# Autodesk Inventor assembly: ALFA1
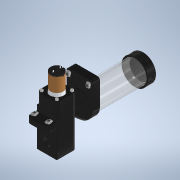
[picture p0: Inventor's stored thumbnail of the model, 180x180]
Saved by Autodesk Inventor 2020.2 (Build 242310000, 310)
## iProperties
Created: 2020-11-09
Part Number: ALFA1
Document SubType Name: Assembly
Designer: JK
Author: JK
## Documents named in this file (15)
- C:\Users\JK\Documents\Inventor\BioMixer\DispensadorPolvo\DispensadordePolvo.iam
- C:\Users\JK\Documents\Inventor\BioMixer\DispensadorPolvo\JGA25-372 24V Motor.ipt
- C:\Users\JK\Documents\Inventor\BioMixer\DispensadorPolvo\Bearing.ipt
- C:\Users\JK\Documents\Inventor\BioMixer\DispensadorPolvo\soportemotor.ipt
- C:\Users\JK\Documents\Inventor\BioMixer\DispensadorPolvo\taparodamiento.ipt
- C:\Users\JK\Documents\Inventor\BioMixer\DispensadorPolvo\TornilloDCGrande.ipt
- C:\Users\JK\Documents\Inventor\BioMixer\DispensadorPolvo\Conjuntocontenedor.iam
- C:\Users\JK\Documents\Inventor\BioMixer\DispensadorPolvo\PernoM5x15Plano.ipt
- C:\Users\JK\Documents\Inventor\BioMixer\DispensadorPolvo\TuercaTM5Perfil2020.ipt
- C:\Users\JK\Documents\Inventor\BioMixer\DispensadorPolvo\BarrilDispensador.ipt
- C:\Users\JK\Documents\Inventor\BioMixer\DispensadorPolvo\PernoM3x6Avellanado.ipt
- C:\Users\JK\Documents\Inventor\BioMixer\DispensadorPolvo\TuercaM3.ipt
- C:\Users\JK\Documents\Inventor\BioMixer\DispensadorPolvo\PernoM3x10Parker.ipt
- C:\Users\JK\Documents\Inventor\BioMixer\DispensadorPolvo\PernoM3x30Parker.ipt
- C:\Users\JK\Documents\Inventor\BioMixer\DispensadorPolvo\PrisioneroM3x6.ipt
## Components (31 placed, 14 different names)
1. JGA25-372 24V Motor:1 — Mate:17, Mate:18, Mate:19, Mate:22, Mate:27, Mate:30, Mate:31, Mate:39, Mate:40, Mate:59
2. BarrilDispensador:1 — Mate:25, Mate:26, Mate:27, Mate:28, Mate:29, Flush:1, Mate:32, Mate:33, Mate:34, Mate:35, Angle:2, Angle:3, Mate:38, Flush:5, Angle:4, Angle:5, Angle:6, Angle:7, Angle:8, Angle:9, Angle:10, Angle:11, Mate:49, Mate:50
3. Bearing:1 — Mate:25, Mate:26
4. soportemotor:1 — Mate:17, Mate:18, Mate:19, Mate:29, Flush:1, Angle:1, Flush:6, Flush:7, Mate:60, Mate:61
5. taparodamiento:1 — Mate:22, Mate:28, Flush:5, Mate:41, Mate:42, Mate:43, Mate:44, Mate:46, Mate:47, Mate:48, Mate:51, Mate:52, Mate:53, Mate:54, Mate:55
6. TornilloDCGrande:1 — Mate:30, Mate:31, Mate:56, Angle:12, Mate:58
7. Conjuntocontenedor:1 [sub-assembly] — Mate:32, Angle:1
8. PernoM5x15Plano:1 — Mate:34, Flush:3, Mate:37
9. PernoM5x15Plano:2 — Mate:33, Flush:3, Mate:35, Mate:36
10. TuercaTM5Perfil2020:1 — Mate:36, Angle:2, Flush:4, Mate:38
11. TuercaTM5Perfil2020:2 — Mate:37, Angle:3, Flush:4
12. PernoM3x6Avellanado:1 — Mate:39, Flush:6
13. PernoM3x6Avellanado:2 — Mate:40, Flush:7
14. TuercaM3:1 — Mate:43, Angle:6, Flush:10
15. TuercaM3:2 — Angle:9, Flush:11, Mate:47, Mate:49
16. TuercaM3:3 — Mate:44, Angle:7, Flush:9, Mate:50
17. TuercaM3:4 — Angle:10, Flush:13, Mate:48
18. TuercaM3:5 — Angle:11, Flush:12, Mate:46
19. TuercaM3:6 — Angle:8, Mate:45, Flush:11, Flush:12, Flush:13
20. TuercaM3:7 — Mate:42, Angle:4, Flush:8
21. TuercaM3:8 — Mate:41, Angle:5, Mate:45, Flush:8, Flush:9, Flush:10
22. PernoM3x10Parker:1 — Mate:51, Mate:52, Flush:14
23. PernoM3x10Parker:2 — Mate:55, Flush:16
24. PernoM3x10Parker:3 — Mate:53, Flush:14, Flush:15
25. PernoM3x10Parker:4 — Mate:54, Flush:15, Flush:16
26. PrisioneroM3x6:1 — Mate:56, Mate:57, Mate:59
27. TuercaM3:9 — Mate:57, Angle:12, Mate:58
28. PernoM3x30Parker:3 — Mate:60, Mate:61
29. PernoM3x30Parker:5
30. PernoM3x30Parker:6
31. PernoM3x30Parker:7
## Component patterns: (4 elements, first: PernoM3x30Parker:3)
## Relationships (68: Mate 41, Flush 15, Angle 12)
- Mate:17: JGA25-372 24V Motor:1 ↔ soportemotor:1
- Mate:18: JGA25-372 24V Motor:1 ↔ soportemotor:1
- Mate:19: JGA25-372 24V Motor:1 ↔ soportemotor:1
- Mate:22: JGA25-372 24V Motor:1 ↔ taparodamiento:1
- Mate:25: BarrilDispensador:1 ↔ Bearing:1
- Mate:26: BarrilDispensador:1 ↔ Bearing:1
- Mate:27: JGA25-372 24V Motor:1 ↔ BarrilDispensador:1
- Mate:28: BarrilDispensador:1 ↔ taparodamiento:1
- Mate:29: BarrilDispensador:1 ↔ soportemotor:1
- Flush:1: BarrilDispensador:1 ↔ soportemotor:1
- Mate:30: JGA25-372 24V Motor:1 ↔ TornilloDCGrande:1
- Mate:31: JGA25-372 24V Motor:1 ↔ TornilloDCGrande:1
- Mate:32: BarrilDispensador:1 ↔ Conjuntocontenedor:1
- Angle:1 (0 deg): soportemotor:1 ↔ Conjuntocontenedor:1
- Mate:33: BarrilDispensador:1 ↔ PernoM5x15Plano:2
- Mate:34: BarrilDispensador:1 ↔ PernoM5x15Plano:1
- Flush:3: PernoM5x15Plano:1 ↔ PernoM5x15Plano:2
- Mate:35: BarrilDispensador:1 ↔ PernoM5x15Plano:2
- Mate:36: PernoM5x15Plano:2 ↔ TuercaTM5Perfil2020:1
- Mate:37: PernoM5x15Plano:1 ↔ TuercaTM5Perfil2020:2
- Angle:2 (0 deg): BarrilDispensador:1 ↔ TuercaTM5Perfil2020:1
- Angle:3 (0 deg): BarrilDispensador:1 ↔ TuercaTM5Perfil2020:2
- Flush:4: TuercaTM5Perfil2020:1 ↔ TuercaTM5Perfil2020:2
- Mate:38 (0.5 mm): BarrilDispensador:1 ↔ TuercaTM5Perfil2020:1
- Flush:5: BarrilDispensador:1 ↔ taparodamiento:1
- Mate:39: JGA25-372 24V Motor:1 ↔ PernoM3x6Avellanado:1
- Flush:6: soportemotor:1 ↔ PernoM3x6Avellanado:1
- Mate:40: JGA25-372 24V Motor:1 ↔ PernoM3x6Avellanado:2
- Flush:7: soportemotor:1 ↔ PernoM3x6Avellanado:2
- Mate:41: taparodamiento:1 ↔ TuercaM3:8
- Mate:42: taparodamiento:1 ↔ TuercaM3:7
- Mate:43: taparodamiento:1 ↔ TuercaM3:1
- Mate:44: taparodamiento:1 ↔ TuercaM3:3
- Angle:4 (0 deg): BarrilDispensador:1 ↔ TuercaM3:7
- Angle:5 (0 deg): BarrilDispensador:1 ↔ TuercaM3:8
- Angle:6 (0 deg): BarrilDispensador:1 ↔ TuercaM3:1
- Angle:7 (0 deg): BarrilDispensador:1 ↔ TuercaM3:3
- Angle:8 (0 deg): BarrilDispensador:1 ↔ TuercaM3:6
- Angle:9 (0 deg): BarrilDispensador:1 ↔ TuercaM3:2
- Angle:10 (0 deg): BarrilDispensador:1 ↔ TuercaM3:4
- Angle:11 (0 deg): BarrilDispensador:1 ↔ TuercaM3:5
- Mate:45: TuercaM3:6 ↔ TuercaM3:8
- Flush:8: TuercaM3:7 ↔ TuercaM3:8
- Flush:9: TuercaM3:3 ↔ TuercaM3:8
- Flush:10: TuercaM3:1 ↔ TuercaM3:8
- Flush:11: TuercaM3:2 ↔ TuercaM3:6
- Flush:12: TuercaM3:5 ↔ TuercaM3:6
- Flush:13: TuercaM3:4 ↔ TuercaM3:6
- Mate:46: taparodamiento:1 ↔ TuercaM3:5
- Mate:47: taparodamiento:1 ↔ TuercaM3:2
- Mate:48: taparodamiento:1 ↔ TuercaM3:4
- Mate:49: BarrilDispensador:1 ↔ TuercaM3:2
- Mate:50: BarrilDispensador:1 ↔ TuercaM3:3
- Mate:51: taparodamiento:1 ↔ PernoM3x10Parker:1
- Mate:52: taparodamiento:1 ↔ PernoM3x10Parker:1
- Mate:53: taparodamiento:1 ↔ PernoM3x10Parker:3
- Mate:54: taparodamiento:1 ↔ PernoM3x10Parker:4
- Mate:55: taparodamiento:1 ↔ PernoM3x10Parker:2
- Flush:14: PernoM3x10Parker:1 ↔ PernoM3x10Parker:3
- Flush:15: PernoM3x10Parker:3 ↔ PernoM3x10Parker:4
- Flush:16: PernoM3x10Parker:2 ↔ PernoM3x10Parker:4
- Mate:56: TornilloDCGrande:1 ↔ PrisioneroM3x6:1
- Mate:57: PrisioneroM3x6:1 ↔ TuercaM3:9
- Angle:12 (0 deg): TornilloDCGrande:1 ↔ TuercaM3:9
- Mate:58: TornilloDCGrande:1 ↔ TuercaM3:9
- Mate:59: JGA25-372 24V Motor:1 ↔ PrisioneroM3x6:1
- Mate:60: soportemotor:1 ↔ PernoM3x30Parker:3
- Mate:61: soportemotor:1 ↔ PernoM3x30Parker:3
